# Autodesk Inventor assembly: Ensamblaje - Base con
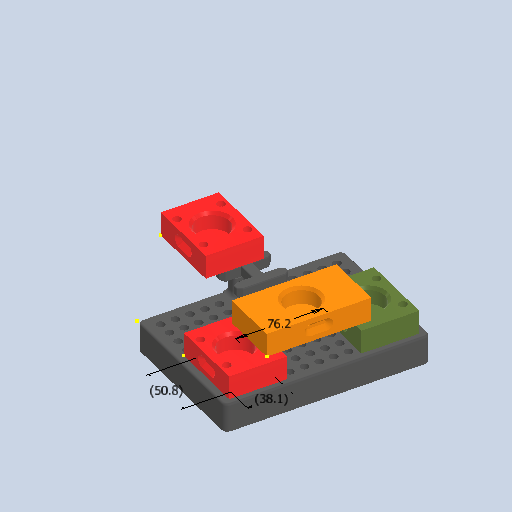
[picture p0: Inventor's stored thumbnail of the model, 512x512]
Saved by Autodesk Inventor 2026 (Build 300175050, 175E)
## iProperties
Created: 2025-09-26
Part Number: Ensamblaje - Base con
Document SubType Name: Assembly
Designer: bello
Author: bello
## Documents named in this file (7)
- A:\Federico Bellomi\UNLZ\5. Quinto Año\PPS\Ensamblaje - Base con Acoples.iam
- A:\Federico Bellomi\UNLZ\5. Quinto Año\PPS\Base.ipt
- A:\Federico Bellomi\UNLZ\5. Quinto Año\PPS\Segundo Acople.ipt
- A:\Federico Bellomi\UNLZ\5. Quinto Año\PPS\Primer Acople.ipt
- A:\Federico Bellomi\UNLZ\5. Quinto Año\PPS\Pieza Izquierda.ipt
- A:\Federico Bellomi\UNLZ\5. Quinto Año\PPS\Pieza Derecha.ipt
- A:\Federico Bellomi\UNLZ\5. Quinto Año\PPS\Pieza Central.ipt
## Components (7 placed, 6 different names)
1. Base:1 — Coincidencia:6, Coincidencia:7, Coincidencia:8, Coincidencia:9, Coincidencia:10, Coincidencia:11, Coincidencia:15, Coincidencia:16, Coincidencia:17
2. Pieza Izquierda:1 — Coincidencia:6, Coincidencia:7, Coincidencia:8, Coincidencia:12
3. Pieza Derecha:1 — Coincidencia:9, Coincidencia:10, Coincidencia:11, Coincidencia:13, Coincidencia:14
4. Primer Acople:1 — Coincidencia:15, Coincidencia:16, Coincidencia:17, Coincidencia:18, Coincidencia:19, Coincidencia:20
5. Segundo Acople:1 — Coincidencia:18, Coincidencia:19, Coincidencia:20
6. Pieza Central:1 — Coincidencia:12, Coincidencia:13, Coincidencia:14
7. Pieza Izquierda:2
## Relationships (15: Mate 15)
- Coincidencia:6 [Mate]: Base:1 ↔ Pieza Izquierda:1
- Coincidencia:7 [Mate]: Base:1 ↔ Pieza Izquierda:1
- Coincidencia:8 [Mate]: Base:1 ↔ Pieza Izquierda:1
- Coincidencia:9 [Mate]: Base:1 ↔ Pieza Derecha:1
- Coincidencia:10 [Mate]: Base:1 ↔ Pieza Derecha:1
- Coincidencia:11 [Mate]: Base:1 ↔ Pieza Derecha:1
- Coincidencia:12 [Mate]: Pieza Izquierda:1 ↔ Pieza Central:1
- Coincidencia:13 [Mate]: Pieza Derecha:1 ↔ Pieza Central:1
- Coincidencia:14 [Mate]: Pieza Derecha:1 ↔ Pieza Central:1
- Coincidencia:15 [Mate]: Base:1 ↔ Primer Acople:1
- Coincidencia:16 [Mate]: Base:1 ↔ Primer Acople:1
- Coincidencia:17 [Mate]: Base:1 ↔ Primer Acople:1
- Coincidencia:18 [Mate]: Primer Acople:1 ↔ Segundo Acople:1
- Coincidencia:19 [Mate]: Primer Acople:1 ↔ Segundo Acople:1
- Coincidencia:20 [Mate]: Primer Acople:1 ↔ Segundo Acople:1
